# Autodesk Inventor assembly: bay_assembly
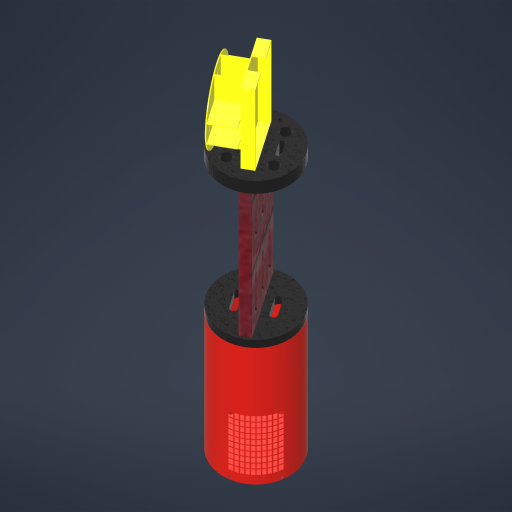
[picture p0: Inventor's stored thumbnail of the model, 512x512]
Saved by Autodesk Inventor 2023 (Build 270158000, 158)
## iProperties
Created: 2022-11-18
Part Number: bay_assembly
Document SubType Name: Assembly
Designer: washington
Author: washington
## Documents named in this file (7)
- C:\Users\washi\Desktop\NAKUJA\N2AvionicsBayDesign\bay_assembly.iam
- C:\Users\washi\Desktop\NAKUJA\N2AvionicsBayDesign\battery_holder_75mm\battery_holder_75mm.ipt
- C:\Users\washi\Desktop\NAKUJA\N2AvionicsBayDesign\bay_bottom_75mm\bay_bottom_75mm.ipt
- C:\Users\washi\Desktop\NAKUJA\N2AvionicsBayDesign\bay_mid_75mm\bay_mid_75mm.ipt
- C:\Users\washi\Desktop\NAKUJA\N2AvionicsBayDesign\bay_top_75mm\bay_top_75mm.ipt
- C:\Users\washi\Desktop\NAKUJA\N2AvionicsBayDesign\pcb\PCB_PCB_N2 Avionics board_2_2022-11-19 PCB.ipt
- C:\Users\washi\Desktop\NAKUJA\N2AvionicsBayDesign\Fin_control_block\Mass.ipt
## Components (6 placed, 6 different names)
1. battery_holder_75mm:1 — Mate:21, Mate:22
2. bay_bottom_75mm:1 — Mate:12, Mate:13, Mate:15, Mate:21, Mate:22
3. bay_mid_75mm:1 — Mate:9, Mate:10, Mate:11, Mate:12, Mate:13, Mate:14, Mate:15, Mate:16, Mate:17, Mate:18
4. bay_top_75mm:1 — Mate:16, Mate:17, Mate:18, Mate:19, Mate:20, Mate:23
5. PCB_PCB_N2 Avionics board_2_2022-11-19 PCB:1 — Mate:9, Mate:10, Mate:11, Mate:14
6. Mass:1 — Mate:19, Mate:20, Mate:23
## Relationships (15: Mate 15)
- Mate:9: bay_mid_75mm:1 ↔ PCB_PCB_N2 Avionics board_2_2022-11-19 PCB:1
- Mate:10: bay_mid_75mm:1 ↔ PCB_PCB_N2 Avionics board_2_2022-11-19 PCB:1
- Mate:11: bay_mid_75mm:1 ↔ PCB_PCB_N2 Avionics board_2_2022-11-19 PCB:1
- Mate:12: bay_bottom_75mm:1 ↔ bay_mid_75mm:1
- Mate:13: bay_bottom_75mm:1 ↔ bay_mid_75mm:1
- Mate:14: bay_mid_75mm:1 ↔ PCB_PCB_N2 Avionics board_2_2022-11-19 PCB:1
- Mate:15: bay_bottom_75mm:1 ↔ bay_mid_75mm:1
- Mate:16: bay_mid_75mm:1 ↔ bay_top_75mm:1
- Mate:17: bay_mid_75mm:1 ↔ bay_top_75mm:1
- Mate:18: bay_mid_75mm:1 ↔ bay_top_75mm:1
- Mate:19: bay_top_75mm:1 ↔ Mass:1
- Mate:20: bay_top_75mm:1 ↔ Mass:1
- Mate:21: battery_holder_75mm:1 ↔ bay_bottom_75mm:1
- Mate:22: battery_holder_75mm:1 ↔ bay_bottom_75mm:1
- Mate:23: bay_top_75mm:1 ↔ Mass:1
